# Autodesk Inventor assembly: BallCatcher
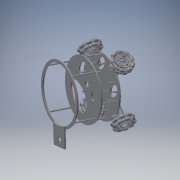
[picture p0: Inventor's stored thumbnail of the model, 180x180]
Saved by Autodesk Inventor 2016 (Build 200138000, 138)
## iProperties
Created: 2016-04-07
Part Number: BallCatcher
Document SubType Name: Assembly
Designer: Ethan
Author: Ethan
## Documents named in this file (16)
- H:\CarLab\Car_Lab_CAD\BallCatcher.iam
- H:\CarLab\Car_Lab_CAD\Base_Acryllic.ipt
- H:\CarLab\Car_Lab_CAD\LBlock.ipt
- H:\CarLab\Car_Lab_CAD\Motor_Mount_Acryllic.ipt
- C:\Users\Ethan\Documents\Inventor\25d-metal-gearmotor-20.4.ipt
- H:\CarLab\Car_Lab_CAD\Motor_Mount_3DPrint.ipt
- H:\CarLab\Car_Lab_CAD\Motor_Hub_Polulu.ipt
- H:\CarLab\Car_Lab_CAD\Imported Components\Vex_Omni_Wheel_4in\Vex_Omni_Wheel_4in.iam
- H:\CarLab\Car_Lab_CAD\Hub_Adapter_Acryllic.ipt
- H:\CarLab\Car_Lab_CAD\Hex_Standoff.ipt
- H:\CarLab\Car_Lab_CAD\Hex_Standoff_CPY.ipt
- H:\CarLab\Car_Lab_CAD\Hex_Standoff_CPY1.ipt
- H:\CarLab\Car_Lab_CAD\Hex_Standoff_CPY_CPY.ipt
- H:\CarLab\Car_Lab_CAD\LayerTwo_Acryllic.ipt
- H:\CarLab\Car_Lab_CAD\Rim_Acryllic.ipt
- H:\CarLab\Car_Lab_CAD\Camera_Mount_Acryllic.ipt
## Components (84 placed, 15 different names)
1. Base_Acryllic:1 — Mate:1, Mate:2, Mate:3, Mate:4, Mate:5, Mate:6, Mate:7, Mate:8, Mate:9, Mate:10, Mate:11, Mate:12, Mate:13, Mate:14, Mate:39, Mate:42, Mate:45, Mate:48, Mate:82, Mate:83, Mate:84, Mate:85, Mate:86, Flush:12, Flush:13, Flush:14, Flush:15, Mate:91, Flush:18, Mate:96, Flush:21, Mate:105, Mate:106, Flush:26, Flush:27, Mate:107, Mate:108, Mate:109, Mate:110, Flush:28, Flush:29, Flush:30, Flush:31, Mate:111, Mate:112, Mate:113, Mate:114, Flush:32, Flush:33, Flush:34, Flush:35, Mate:115, Mate:116, Mate:117, Mate:118, Flush:36, Flush:37, Flush:38, Flush:39, Mate:119, Mate:120, Mate:121, Mate:122, Flush:40, Flush:41, Flush:42, Flush:43
2. LBlock:1 — Mate:1, Mate:2, Flush:1, Mate:20
3. LBlock:2 — Flush:1, Mate:3, Mate:4, Mate:18, Mate:19
4. LBlock:3 — Mate:5, Mate:6, Flush:5, Mate:22, Mate:23
5. LBlock:4 — Mate:7, Mate:8, Flush:5, Mate:21
6. LBlock:5 — Mate:10, Flush:3, Flush:4, Mate:24, Mate:26
7. LBlock:6 — Mate:9, Flush:3, Flush:4, Mate:11, Mate:25
8. LBlock:7 — Mate:13, Flush:6, Flush:7, Mate:15, Mate:16
9. LBlock:8 — Mate:12, Flush:6, Flush:7, Mate:14, Mate:17
10. Motor_Mount_Acryllic:1 — Mate:21, Mate:22, Mate:23, Mate:30, Mate:31, Mate:32
11. Motor_Mount_Acryllic:2 — Mate:18, Mate:19, Mate:20, Mate:36, Mate:37, Mate:38
12. Motor_Mount_Acryllic:3 — Mate:24, Mate:25, Mate:26, Mate:27, Mate:28, Mate:29
13. Motor_Mount_Acryllic:4 — Mate:15, Mate:16, Mate:17, Mate:33, Mate:34, Mate:35
14. 25d-metal-gearmotor-20.4:1 — Mate:27, Mate:28, Mate:29, Mate:46, Mate:47, Flush:8, Mate:51
15. 25d-metal-gearmotor-20.4:2 — Mate:33, Mate:34, Mate:35, Mate:40, Mate:41, Flush:10, Mate:53
16. 25d-metal-gearmotor-20.4:3 — Mate:36, Mate:37, Mate:38, Mate:49, Mate:50, Flush:11, Mate:54
17. 25d-metal-gearmotor-20.4:4 — Mate:30, Mate:31, Mate:32, Mate:43, Mate:44, Flush:9, Mate:52
18. Motor_Mount_3DPrint:1 — Mate:45, Mate:46, Mate:47
19. Motor_Mount_3DPrint:2 — Mate:42, Mate:43, Mate:44
20. Motor_Mount_3DPrint:3 — Mate:39, Mate:40, Mate:41
21. Motor_Mount_3DPrint:4 — Mate:48, Mate:49, Mate:50
22. Motor_Hub_Polulu:1 — Flush:10, Mate:53, Mate:75, Mate:76, Mate:78
23. Motor_Hub_Polulu:2 — Flush:11, Mate:54, Mate:69, Mate:70, Mate:71
24. Motor_Hub_Polulu:3 — Flush:9, Mate:52, Mate:62, Mate:64, Mate:65
25. Motor_Hub_Polulu:4 — Flush:8, Mate:51, Mate:59, Mate:60, Mate:61
26. Vex_Omni_Wheel_4in:1 [sub-assembly] — Mate:55, Mate:56, Mate:57, Mate:58
27. Vex_Omni_Wheel_4in:2 [sub-assembly] — Mate:66, Mate:67, Mate:68
28. Vex_Omni_Wheel_4in:3 [sub-assembly] — Mate:72, Mate:73, Mate:74
29. Vex_Omni_Wheel_4in:4 [sub-assembly] — Mate:77, Mate:79, Mate:80, Mate:81
30. Hub_Adapter_Acryllic:1 — Mate:69, Mate:70, Mate:71, Mate:72, Mate:73, Mate:74
31. Hub_Adapter_Acryllic:2 — Mate:75, Mate:76, Mate:77, Mate:78, Mate:79, Mate:80, Mate:81
32. Hub_Adapter_Acryllic:3 — Mate:62, Mate:64, Mate:65, Mate:66, Mate:67, Mate:68
33. Hub_Adapter_Acryllic:4 — Mate:55, Mate:56, Mate:57, Mate:58, Mate:59, Mate:60, Mate:61
34. Hex_Standoff:1 — Mate:87, Flush:17, Mate:90, Mate:91, Flush:18
35. Hex_Standoff:2 — Mate:87, Mate:88, Flush:16, Flush:17, Mate:89, Mate:90
36. Hex_Standoff:3 — Mate:84, Flush:15
37. Hex_Standoff:4 — Mate:82, Mate:83, Flush:14
38. Hex_Standoff:5 — Mate:88, Flush:16, Mate:89, Mate:147
39. Hex_Standoff:6 — Mate:85, Flush:13
40. Hex_Standoff:7 — Mate:86, Flush:12
41. Hex_Standoff_CPY:1 — Mate:92, Flush:19, Mate:93, Mate:96, Flush:21
42. Hex_Standoff_CPY:2 — Mate:92, Flush:19, Mate:93, Mate:94, Flush:20, Mate:95
43. Hex_Standoff_CPY:3 — Mate:94, Flush:20, Mate:95, Mate:148
44. Hex_Standoff_CPY1:1 — Mate:97, Flush:22, Mate:98, Flush:27
45. Hex_Standoff_CPY1:2 — Mate:97, Flush:22, Mate:98, Mate:99, Flush:23, Mate:100
46. Hex_Standoff_CPY1:3 — Mate:99, Flush:23, Mate:100, Mate:105, Mate:150
47. Hex_Standoff_CPY_CPY:1 — Mate:101, Flush:24, Mate:102, Flush:26
48. Hex_Standoff_CPY_CPY:2 — Mate:101, Flush:24, Mate:102, Mate:103, Flush:25, Mate:104
49. Hex_Standoff_CPY_CPY:3 — Mate:103, Flush:25, Mate:104, Mate:106, Mate:149
50. Hex_Standoff:8 — Mate:108, Flush:28
51. Hex_Standoff:9 — Mate:107, Flush:29
52. Hex_Standoff:10 — Mate:109, Flush:30
53. Hex_Standoff:11 — Mate:110, Flush:31
54. Hex_Standoff:12 — Mate:111, Flush:32
55. Hex_Standoff:13 — Mate:112, Flush:35
56. Hex_Standoff:14 — Mate:114, Flush:33
57. Hex_Standoff:15 — Mate:113, Flush:34
58. Hex_Standoff:16 — Mate:115, Flush:39
59. Hex_Standoff:17 — Mate:116, Flush:37
60. Hex_Standoff:18 — Mate:117, Flush:36
61. Hex_Standoff:19 — Mate:118, Flush:38
62. Hex_Standoff:20 — Mate:120, Flush:41
63. Hex_Standoff:21 — Mate:119, Flush:43
64. Hex_Standoff:22 — Mate:121, Flush:42
65. Hex_Standoff:23 — Mate:122, Flush:40
66. Hex_Standoff_CPY1:4 — Flush:54, Mate:151, Mate:152
67. Hex_Standoff_CPY1:5
68. Hex_Standoff_CPY1:6 — Mate:127, Mate:128
69. Hex_Standoff_CPY1:7 — Mate:127, Mate:128, Mate:158
70. Hex_Standoff_CPY1:8 — Flush:53, Flush:54, Mate:155
71. Hex_Standoff_CPY1:9
72. Hex_Standoff_CPY1:10
73. Hex_Standoff_CPY1:11 — Mate:160, Mate:163, Mate:166, Mate:167
74. Hex_Standoff_CPY1:12 — Flush:52, Flush:53, Mate:154
75. Hex_Standoff_CPY1:13
76. Hex_Standoff_CPY1:14
77. Hex_Standoff_CPY1:15 — Mate:157, Mate:159, Mate:161, Mate:162, Mate:164, Mate:165
78. Hex_Standoff_CPY1:16 — Flush:52, Mate:153
79. Hex_Standoff_CPY1:17
80. Hex_Standoff_CPY1:18
81. Hex_Standoff_CPY1:19 — Mate:156
82. LayerTwo_Acryllic:1 — Mate:147, Mate:148, Mate:149, Mate:150, Mate:151, Mate:152, Mate:153, Mate:154, Mate:155
83. Rim_Acryllic:1 — Mate:156, Mate:157, Mate:158, Mate:159, Mate:160, Mate:161, Mate:162, Mate:163, Mate:164, Mate:165, Mate:166, Mate:167, Mate:168, Mate:169, Mate:170
84. Camera_Mount_Acryllic:1 — Mate:168, Mate:169, Mate:170
## Relationships (222: Mate 169, Flush 53)
- Mate:1: Base_Acryllic:1 ↔ LBlock:1
- Mate:2: Base_Acryllic:1 ↔ LBlock:1
- Flush:1: LBlock:1 ↔ LBlock:2
- Mate:3: Base_Acryllic:1 ↔ LBlock:2
- Mate:4: Base_Acryllic:1 ↔ LBlock:2
- Mate:5: Base_Acryllic:1 ↔ LBlock:3
- Mate:6: Base_Acryllic:1 ↔ LBlock:3
- Mate:7: Base_Acryllic:1 ↔ LBlock:4
- Mate:8: Base_Acryllic:1 ↔ LBlock:4
- Mate:9: Base_Acryllic:1 ↔ LBlock:6
- Mate:10: Base_Acryllic:1 ↔ LBlock:5
- Flush:3: LBlock:5 ↔ LBlock:6
- Flush:4: LBlock:5 ↔ LBlock:6
- Mate:11: Base_Acryllic:1 ↔ LBlock:6
- Flush:5: LBlock:3 ↔ LBlock:4
- Mate:12: Base_Acryllic:1 ↔ LBlock:8
- Mate:13: Base_Acryllic:1 ↔ LBlock:7
- Flush:6: LBlock:7 ↔ LBlock:8
- Flush:7: LBlock:7 ↔ LBlock:8
- Mate:14: Base_Acryllic:1 ↔ LBlock:8
- Mate:15: LBlock:7 ↔ Motor_Mount_Acryllic:4
- Mate:16: LBlock:7 ↔ Motor_Mount_Acryllic:4
- Mate:17: LBlock:8 ↔ Motor_Mount_Acryllic:4
- Mate:18: LBlock:2 ↔ Motor_Mount_Acryllic:2
- Mate:19: LBlock:2 ↔ Motor_Mount_Acryllic:2
- Mate:20: LBlock:1 ↔ Motor_Mount_Acryllic:2
- Mate:21: LBlock:4 ↔ Motor_Mount_Acryllic:1
- Mate:22: LBlock:3 ↔ Motor_Mount_Acryllic:1
- Mate:23: LBlock:3 ↔ Motor_Mount_Acryllic:1
- Mate:24: LBlock:5 ↔ Motor_Mount_Acryllic:3
- Mate:25: LBlock:6 ↔ Motor_Mount_Acryllic:3
- Mate:26: LBlock:5 ↔ Motor_Mount_Acryllic:3
- Mate:27: Motor_Mount_Acryllic:3 ↔ 25d-metal-gearmotor-20.4:1
- Mate:28: Motor_Mount_Acryllic:3 ↔ 25d-metal-gearmotor-20.4:1
- Mate:29: Motor_Mount_Acryllic:3 ↔ 25d-metal-gearmotor-20.4:1
- Mate:30: Motor_Mount_Acryllic:1 ↔ 25d-metal-gearmotor-20.4:4
- Mate:31: Motor_Mount_Acryllic:1 ↔ 25d-metal-gearmotor-20.4:4
- Mate:32: Motor_Mount_Acryllic:1 ↔ 25d-metal-gearmotor-20.4:4
- Mate:33: Motor_Mount_Acryllic:4 ↔ 25d-metal-gearmotor-20.4:2
- Mate:34: Motor_Mount_Acryllic:4 ↔ 25d-metal-gearmotor-20.4:2
- Mate:35: Motor_Mount_Acryllic:4 ↔ 25d-metal-gearmotor-20.4:2
- Mate:36: Motor_Mount_Acryllic:2 ↔ 25d-metal-gearmotor-20.4:3
- Mate:37: Motor_Mount_Acryllic:2 ↔ 25d-metal-gearmotor-20.4:3
- Mate:38: Motor_Mount_Acryllic:2 ↔ 25d-metal-gearmotor-20.4:3
- Mate:39: Base_Acryllic:1 ↔ Motor_Mount_3DPrint:3
- Mate:40: 25d-metal-gearmotor-20.4:2 ↔ Motor_Mount_3DPrint:3
- Mate:41: 25d-metal-gearmotor-20.4:2 ↔ Motor_Mount_3DPrint:3
- Mate:42: Base_Acryllic:1 ↔ Motor_Mount_3DPrint:2
- Mate:43: 25d-metal-gearmotor-20.4:4 ↔ Motor_Mount_3DPrint:2
- Mate:44: 25d-metal-gearmotor-20.4:4 ↔ Motor_Mount_3DPrint:2
- Mate:45: Base_Acryllic:1 ↔ Motor_Mount_3DPrint:1
- Mate:46: 25d-metal-gearmotor-20.4:1 ↔ Motor_Mount_3DPrint:1
- Mate:47: 25d-metal-gearmotor-20.4:1 ↔ Motor_Mount_3DPrint:1
- Mate:48: Base_Acryllic:1 ↔ Motor_Mount_3DPrint:4
- Mate:49: 25d-metal-gearmotor-20.4:3 ↔ Motor_Mount_3DPrint:4
- Mate:50: 25d-metal-gearmotor-20.4:3 ↔ Motor_Mount_3DPrint:4
- Flush:8: 25d-metal-gearmotor-20.4:1 ↔ Motor_Hub_Polulu:4
- Mate:51: 25d-metal-gearmotor-20.4:1 ↔ Motor_Hub_Polulu:4
- Flush:9: 25d-metal-gearmotor-20.4:4 ↔ Motor_Hub_Polulu:3
- Mate:52: 25d-metal-gearmotor-20.4:4 ↔ Motor_Hub_Polulu:3
- Flush:10: 25d-metal-gearmotor-20.4:2 ↔ Motor_Hub_Polulu:1
- Mate:53: 25d-metal-gearmotor-20.4:2 ↔ Motor_Hub_Polulu:1
- Flush:11: 25d-metal-gearmotor-20.4:3 ↔ Motor_Hub_Polulu:2
- Mate:54: 25d-metal-gearmotor-20.4:3 ↔ Motor_Hub_Polulu:2
- Mate:55: Vex_Omni_Wheel_4in:1 ↔ Hub_Adapter_Acryllic:4
- Mate:56: Vex_Omni_Wheel_4in:1 ↔ Hub_Adapter_Acryllic:4
- Mate:57: Vex_Omni_Wheel_4in:1 ↔ Hub_Adapter_Acryllic:4
- Mate:58: Vex_Omni_Wheel_4in:1 ↔ Hub_Adapter_Acryllic:4
- Mate:59: Motor_Hub_Polulu:4 ↔ Hub_Adapter_Acryllic:4
- Mate:60: Motor_Hub_Polulu:4 ↔ Hub_Adapter_Acryllic:4
- Mate:61: Motor_Hub_Polulu:4 ↔ Hub_Adapter_Acryllic:4
- Mate:62: Motor_Hub_Polulu:3 ↔ Hub_Adapter_Acryllic:3
- Mate:64: Motor_Hub_Polulu:3 ↔ Hub_Adapter_Acryllic:3
- Mate:65: Motor_Hub_Polulu:3 ↔ Hub_Adapter_Acryllic:3
- Mate:66: Vex_Omni_Wheel_4in:2 ↔ Hub_Adapter_Acryllic:3
- Mate:67: Vex_Omni_Wheel_4in:2 ↔ Hub_Adapter_Acryllic:3
- Mate:68: Vex_Omni_Wheel_4in:2 ↔ Hub_Adapter_Acryllic:3
- Mate:69: Motor_Hub_Polulu:2 ↔ Hub_Adapter_Acryllic:1
- Mate:70: Motor_Hub_Polulu:2 ↔ Hub_Adapter_Acryllic:1
- Mate:71: Motor_Hub_Polulu:2 ↔ Hub_Adapter_Acryllic:1
- Mate:72: Vex_Omni_Wheel_4in:3 ↔ Hub_Adapter_Acryllic:1
- Mate:73: Vex_Omni_Wheel_4in:3 ↔ Hub_Adapter_Acryllic:1
- Mate:74: Vex_Omni_Wheel_4in:3 ↔ Hub_Adapter_Acryllic:1
- Mate:75: Motor_Hub_Polulu:1 ↔ Hub_Adapter_Acryllic:2
- Mate:76: Motor_Hub_Polulu:1 ↔ Hub_Adapter_Acryllic:2
- Mate:77: Vex_Omni_Wheel_4in:4 ↔ Hub_Adapter_Acryllic:2
- Mate:78: Motor_Hub_Polulu:1 ↔ Hub_Adapter_Acryllic:2
- Mate:79: Vex_Omni_Wheel_4in:4 ↔ Hub_Adapter_Acryllic:2
- Mate:80: Vex_Omni_Wheel_4in:4 ↔ Hub_Adapter_Acryllic:2
- Mate:81: Vex_Omni_Wheel_4in:4 ↔ Hub_Adapter_Acryllic:2
- Mate:82: Base_Acryllic:1 ↔ Hex_Standoff:4
- Mate:83: Base_Acryllic:1 ↔ Hex_Standoff:4
- Mate:84: Base_Acryllic:1 ↔ Hex_Standoff:3
- Mate:85: Base_Acryllic:1 ↔ Hex_Standoff:6
- Mate:86: Base_Acryllic:1 ↔ Hex_Standoff:7
- Flush:12: Base_Acryllic:1 ↔ Hex_Standoff:7
- Flush:13: Base_Acryllic:1 ↔ Hex_Standoff:6
- Flush:14: Base_Acryllic:1 ↔ Hex_Standoff:4
- Flush:15: Base_Acryllic:1 ↔ Hex_Standoff:3
- Mate:87: Hex_Standoff:1 ↔ Hex_Standoff:2
- Mate:88: Hex_Standoff:2 ↔ Hex_Standoff:5
- Flush:16: Hex_Standoff:2 ↔ Hex_Standoff:5
- Flush:17: Hex_Standoff:1 ↔ Hex_Standoff:2
- Mate:89: Hex_Standoff:2 ↔ Hex_Standoff:5
- Mate:90: Hex_Standoff:1 ↔ Hex_Standoff:2
- Mate:91: Base_Acryllic:1 ↔ Hex_Standoff:1
- Flush:18: Base_Acryllic:1 ↔ Hex_Standoff:1
- Mate:92: Hex_Standoff_CPY:1 ↔ Hex_Standoff_CPY:2
- Flush:19: Hex_Standoff_CPY:1 ↔ Hex_Standoff_CPY:2
- Mate:93: Hex_Standoff_CPY:1 ↔ Hex_Standoff_CPY:2
- Mate:94: Hex_Standoff_CPY:2 ↔ Hex_Standoff_CPY:3
- Flush:20: Hex_Standoff_CPY:2 ↔ Hex_Standoff_CPY:3
- Mate:95: Hex_Standoff_CPY:2 ↔ Hex_Standoff_CPY:3
- Mate:96: Base_Acryllic:1 ↔ Hex_Standoff_CPY:1
- Flush:21: Base_Acryllic:1 ↔ Hex_Standoff_CPY:1
- Mate:97: Hex_Standoff_CPY1:1 ↔ Hex_Standoff_CPY1:2
- Flush:22: Hex_Standoff_CPY1:1 ↔ Hex_Standoff_CPY1:2
- Mate:98: Hex_Standoff_CPY1:1 ↔ Hex_Standoff_CPY1:2
- Mate:99: Hex_Standoff_CPY1:2 ↔ Hex_Standoff_CPY1:3
- Flush:23: Hex_Standoff_CPY1:2 ↔ Hex_Standoff_CPY1:3
- Mate:100: Hex_Standoff_CPY1:2 ↔ Hex_Standoff_CPY1:3
- Mate:101: Hex_Standoff_CPY_CPY:1 ↔ Hex_Standoff_CPY_CPY:2
- Flush:24: Hex_Standoff_CPY_CPY:1 ↔ Hex_Standoff_CPY_CPY:2
- Mate:102: Hex_Standoff_CPY_CPY:1 ↔ Hex_Standoff_CPY_CPY:2
- Mate:103: Hex_Standoff_CPY_CPY:2 ↔ Hex_Standoff_CPY_CPY:3
- Flush:25: Hex_Standoff_CPY_CPY:2 ↔ Hex_Standoff_CPY_CPY:3
- Mate:104: Hex_Standoff_CPY_CPY:2 ↔ Hex_Standoff_CPY_CPY:3
- Mate:105: Base_Acryllic:1 ↔ Hex_Standoff_CPY1:3
- Mate:106: Base_Acryllic:1 ↔ Hex_Standoff_CPY_CPY:3
- Flush:26: Base_Acryllic:1 ↔ Hex_Standoff_CPY_CPY:1
- Flush:27: Base_Acryllic:1 ↔ Hex_Standoff_CPY1:1
- Mate:107: Base_Acryllic:1 ↔ Hex_Standoff:9
- Mate:108: Base_Acryllic:1 ↔ Hex_Standoff:8
- Mate:109: Base_Acryllic:1 ↔ Hex_Standoff:10
- Mate:110: Base_Acryllic:1 ↔ Hex_Standoff:11
- Flush:28: Base_Acryllic:1 ↔ Hex_Standoff:8
- Flush:29: Base_Acryllic:1 ↔ Hex_Standoff:9
- Flush:30: Base_Acryllic:1 ↔ Hex_Standoff:10
- Flush:31: Base_Acryllic:1 ↔ Hex_Standoff:11
- Mate:111: Base_Acryllic:1 ↔ Hex_Standoff:12
- Mate:112: Base_Acryllic:1 ↔ Hex_Standoff:13
- Mate:113: Base_Acryllic:1 ↔ Hex_Standoff:15
- Mate:114: Base_Acryllic:1 ↔ Hex_Standoff:14
- Flush:32: Base_Acryllic:1 ↔ Hex_Standoff:12
- Flush:33: Base_Acryllic:1 ↔ Hex_Standoff:14
- Flush:34: Base_Acryllic:1 ↔ Hex_Standoff:15
- Flush:35: Base_Acryllic:1 ↔ Hex_Standoff:13
- Mate:115: Base_Acryllic:1 ↔ Hex_Standoff:16
- Mate:116: Base_Acryllic:1 ↔ Hex_Standoff:17
- Mate:117: Base_Acryllic:1 ↔ Hex_Standoff:18
- Mate:118: Base_Acryllic:1 ↔ Hex_Standoff:19
- Flush:36: Base_Acryllic:1 ↔ Hex_Standoff:18
- Flush:37: Base_Acryllic:1 ↔ Hex_Standoff:17
- Flush:38: Base_Acryllic:1 ↔ Hex_Standoff:19
- Flush:39: Base_Acryllic:1 ↔ Hex_Standoff:16
- Mate:119: Base_Acryllic:1 ↔ Hex_Standoff:21
- Mate:120: Base_Acryllic:1 ↔ Hex_Standoff:20
- Mate:121: Base_Acryllic:1 ↔ Hex_Standoff:22
- Mate:122: Base_Acryllic:1 ↔ Hex_Standoff:23
- Flush:40: Base_Acryllic:1 ↔ Hex_Standoff:23
- Flush:41: Base_Acryllic:1 ↔ Hex_Standoff:20
- Flush:42: Base_Acryllic:1 ↔ Hex_Standoff:22
- Flush:43: Base_Acryllic:1 ↔ Hex_Standoff:21
- [Mate]: Hex_Standoff_CPY1:4 ↔ Hex_Standoff_CPY1:5
- [Flush]: Hex_Standoff_CPY1:4 ↔ Hex_Standoff_CPY1:5
- [Mate]: Hex_Standoff_CPY1:4 ↔ Hex_Standoff_CPY1:5
- [Mate]: Hex_Standoff_CPY1:5 ↔ Hex_Standoff_CPY1:6
- [Flush]: Hex_Standoff_CPY1:5 ↔ Hex_Standoff_CPY1:6
- [Mate]: Hex_Standoff_CPY1:5 ↔ Hex_Standoff_CPY1:6
- Mate:127: Hex_Standoff_CPY1:6 ↔ Hex_Standoff_CPY1:7
- Mate:128: Hex_Standoff_CPY1:6 ↔ Hex_Standoff_CPY1:7
- [Mate]: Hex_Standoff_CPY1:8 ↔ Hex_Standoff_CPY1:9
- [Flush]: Hex_Standoff_CPY1:8 ↔ Hex_Standoff_CPY1:9
- [Mate]: Hex_Standoff_CPY1:8 ↔ Hex_Standoff_CPY1:9
- [Mate]: Hex_Standoff_CPY1:9 ↔ Hex_Standoff_CPY1:10
- [Flush]: Hex_Standoff_CPY1:9 ↔ Hex_Standoff_CPY1:10
- [Mate]: Hex_Standoff_CPY1:9 ↔ Hex_Standoff_CPY1:10
- [Mate]: Hex_Standoff_CPY1:10 ↔ Hex_Standoff_CPY1:11
- [Mate]: Hex_Standoff_CPY1:10 ↔ Hex_Standoff_CPY1:11
- [Mate]: Hex_Standoff_CPY1:12 ↔ Hex_Standoff_CPY1:13
- [Flush]: Hex_Standoff_CPY1:12 ↔ Hex_Standoff_CPY1:13
- [Mate]: Hex_Standoff_CPY1:12 ↔ Hex_Standoff_CPY1:13
- [Mate]: Hex_Standoff_CPY1:13 ↔ Hex_Standoff_CPY1:14
- [Flush]: Hex_Standoff_CPY1:13 ↔ Hex_Standoff_CPY1:14
- [Mate]: Hex_Standoff_CPY1:13 ↔ Hex_Standoff_CPY1:14
- [Mate]: Hex_Standoff_CPY1:14 ↔ Hex_Standoff_CPY1:15
- [Mate]: Hex_Standoff_CPY1:14 ↔ Hex_Standoff_CPY1:15
- [Mate]: Hex_Standoff_CPY1:16 ↔ Hex_Standoff_CPY1:17
- [Flush]: Hex_Standoff_CPY1:16 ↔ Hex_Standoff_CPY1:17
- [Mate]: Hex_Standoff_CPY1:16 ↔ Hex_Standoff_CPY1:17
- [Mate]: Hex_Standoff_CPY1:17 ↔ Hex_Standoff_CPY1:18
- [Flush]: Hex_Standoff_CPY1:17 ↔ Hex_Standoff_CPY1:18
- [Mate]: Hex_Standoff_CPY1:17 ↔ Hex_Standoff_CPY1:18
- [Mate]: Hex_Standoff_CPY1:18 ↔ Hex_Standoff_CPY1:19
- [Mate]: Hex_Standoff_CPY1:18 ↔ Hex_Standoff_CPY1:19
- Mate:147: Hex_Standoff:5 ↔ LayerTwo_Acryllic:1
- Mate:148: Hex_Standoff_CPY:3 ↔ LayerTwo_Acryllic:1
- Mate:149: Hex_Standoff_CPY_CPY:3 ↔ LayerTwo_Acryllic:1
- Mate:150: Hex_Standoff_CPY1:3 ↔ LayerTwo_Acryllic:1
- Flush:52: Hex_Standoff_CPY1:12 ↔ Hex_Standoff_CPY1:16
- Flush:53: Hex_Standoff_CPY1:8 ↔ Hex_Standoff_CPY1:12
- Flush:54: Hex_Standoff_CPY1:4 ↔ Hex_Standoff_CPY1:8
- Mate:151: Hex_Standoff_CPY1:4 ↔ LayerTwo_Acryllic:1
- Mate:152: Hex_Standoff_CPY1:4 ↔ LayerTwo_Acryllic:1
- Mate:153: Hex_Standoff_CPY1:16 ↔ LayerTwo_Acryllic:1
- Mate:154: Hex_Standoff_CPY1:12 ↔ LayerTwo_Acryllic:1
- Mate:155: Hex_Standoff_CPY1:8 ↔ LayerTwo_Acryllic:1
- Mate:156: Hex_Standoff_CPY1:19 ↔ Rim_Acryllic:1
- Mate:157: Hex_Standoff_CPY1:15 ↔ Rim_Acryllic:1
- Mate:158: Hex_Standoff_CPY1:7 ↔ Rim_Acryllic:1
- Mate:159: Hex_Standoff_CPY1:15 ↔ Rim_Acryllic:1
- Mate:160: Hex_Standoff_CPY1:11 ↔ Rim_Acryllic:1
- Mate:161: Hex_Standoff_CPY1:15 ↔ Rim_Acryllic:1
- Mate:162: Hex_Standoff_CPY1:15 ↔ Rim_Acryllic:1
- Mate:163: Hex_Standoff_CPY1:11 ↔ Rim_Acryllic:1
- Mate:164: Hex_Standoff_CPY1:15 ↔ Rim_Acryllic:1
- Mate:165: Hex_Standoff_CPY1:15 ↔ Rim_Acryllic:1
- Mate:166: Hex_Standoff_CPY1:11 ↔ Rim_Acryllic:1
- Mate:167: Hex_Standoff_CPY1:11 ↔ Rim_Acryllic:1
- Mate:168: Rim_Acryllic:1 ↔ Camera_Mount_Acryllic:1
- Mate:169: Rim_Acryllic:1 ↔ Camera_Mount_Acryllic:1
- Mate:170: Rim_Acryllic:1 ↔ Camera_Mount_Acryllic:1
## Named parameters: d173_d117 = 0 mm, d174_d118 = 0 mm, d175_d119 = 0 mm, d176_d120 = 0 mm, d177_d121 = 0 mm, d178_d122 = 0 mm, d181_d173_d117 = 0 mm, d182_d174_d118 = 0 mm, d183_d175_d119 = 0 mm, d184_d176_d120 = 0 mm, d185_d177_d121 = 0 mm, d186_d178_d122 = 0 mm, d187_d179 = 0 mm, d188_d180 = 0 mm, d189_d173_d117 = 0 mm, d190_d174_d118 = 0 mm, d191_d175_d119 = 0 mm, d192_d176_d120 = 0 mm, d193_d177_d121 = 0 mm, d194_d178_d122 = 0 mm, d195_d179 = 0 mm, d196_d180 = 0 mm, d197_d173_d117 = 0 mm, d198_d174_d118 = 0 mm, d199_d175_d119 = 0 mm, d200_d176_d120 = 0 mm, d201_d177_d121 = 0 mm, d202_d178_d122 = 0 mm, d203_d179 = 0 mm, d204_d180 = 0 mm
